# Autodesk Inventor assembly: Assembly1
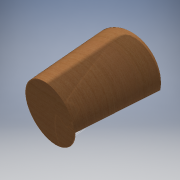
[picture p0: Inventor's stored thumbnail of the model, 180x180]
Saved by Autodesk Inventor 2017.3 (Build 213257000, 257)
## iProperties
Created: 2020-01-20
Part Number: Assembly1
Document SubType Name: Assembly
Designer: Ole Simmering
Author: Ole Simmering
## Documents named in this file (4)
- C:\Users\Ole Simmering\Documents\GitHub\3D_modeling\BWL\Assembly1.iam
- C:\Users\Ole Simmering\Documents\GitHub\3D_modeling\BWL\Elektronik.ipt
- C:\Users\Ole Simmering\Documents\GitHub\3D_modeling\BWL\Tank.ipt
- C:\Users\Ole Simmering\Documents\GitHub\3D_modeling\BWL\Topf.ipt
## Components (3 placed, 3 different names)
1. Elektronik:1 — Mate:1, Mate:2
2. Tank:1 — Mate:1, Mate:2, Mate:3, Mate:4
3. Topf:1 — Mate:3, Mate:4, Mate:5
## Relationships (5: Mate 5)
- Mate:1: Elektronik:1 ↔ Tank:1
- Mate:2: Elektronik:1 ↔ Tank:1
- Mate:3: Tank:1 ↔ Topf:1
- Mate:4 (0.01 mm): Tank:1 ↔ Topf:1
- Mate:5: Topf:1
